# Autodesk Inventor assembly: AM14U5_LONG_TOUGHBOX_MINI_6IN_H_ASM
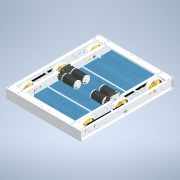
[picture p0: Inventor's stored thumbnail of the model, 180x180]
Saved by Autodesk Inventor 2022.2 (Build 262287000, 287)
## iProperties
Created: 2022-01-21
Part Number: AM14U5_LONG_TOUGHBOX_MINI_6IN_H_ASM
Document SubType Name: Assembly
Designer: robst
Author: robst
Revision Number: 9LAST_VERSION
## Documents named in this file (4)
- C:\git\CAD-Development\robSteele\2022 Robot\EveryBot\AM14U5_LONG_TOUGHBOX_MINI_6IN_H_ASM.iam
- C:\git\CAD-Development\robSteele\2022 Robot\EveryBot\AM14U5_LONG_TOUGHBOX_MINI_6IN_1_ASM.iam
- C:\git\CAD-Development\robSteele\2022 Robot\EveryBot\3_375IN_CHURRO.ipt
- C:\git\CAD-Development\robSteele\2022 Robot\EveryBot\PlywoodBasePlate17_25x32_03x0_5inches.ipt
## Components (4 placed, 4 different names)
1. 828 [sub-assembly] — Mate:1, Mate:2, Mate:3
2. 829
3. 830
4. PlywoodBasePlate17_25x32_03x0_5inches:1 — Mate:1, Mate:2, Mate:3
## Relationships (3: Mate 3)
- Mate:1: 828 ↔ PlywoodBasePlate17_25x32_03x0_5inches:1
- Mate:2: 828 ↔ PlywoodBasePlate17_25x32_03x0_5inches:1
- Mate:3: 828 ↔ PlywoodBasePlate17_25x32_03x0_5inches:1
